# Autodesk Inventor assembly: Assembly1
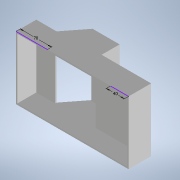
[picture p0: Inventor's stored thumbnail of the model, 180x180]
Saved by Autodesk Inventor 2022 (Build 260153000, 153)
## iProperties
Created: 2021-12-16
Part Number: Assembly1
Document SubType Name: Assembly
Designer: keemi
Author: keemi
## Documents named in this file (9)
- C:\Users\keemi\OneDrive\Bureaublad\repo's\projecten\Auto\modellen\inventor\auto moddel\Assembly1.iam
- C:\Users\keemi\OneDrive\Bureaublad\repo's\projecten\Auto\modellen\inventor\auto moddel\zijkant.ipt
- C:\Users\keemi\OneDrive\Bureaublad\repo's\projecten\Auto\modellen\inventor\auto moddel\onderkant.ipt
- C:\Users\keemi\OneDrive\Bureaublad\repo's\projecten\Auto\modellen\inventor\auto moddel\voorkant.ipt
- C:\Users\keemi\OneDrive\Bureaublad\repo's\projecten\Auto\modellen\inventor\auto moddel\achterkant.ipt
- C:\Users\keemi\OneDrive\Bureaublad\repo's\projecten\Auto\modellen\inventor\auto moddel\motorkap.ipt
- C:\Users\keemi\OneDrive\Bureaublad\repo's\projecten\Auto\modellen\inventor\auto moddel\achterruit.ipt
- C:\Users\keemi\OneDrive\Bureaublad\repo's\projecten\Auto\modellen\inventor\auto moddel\bak.ipt
- C:\Users\keemi\OneDrive\Bureaublad\repo's\projecten\Auto\modellen\inventor\auto moddel\DAK.ipt
## Components (9 placed, 8 different names)
1. zijkant:1 — Flush:11, Flush:12, Flush:13, Flush:14, Flush:15, Flush:16, Flush:18, Flush:20, Flush:24
2. onderkant:1 — Flush:3, Flush:4, Flush:5, Flush:8, Flush:11, Flush:12
3. zijkant:2 — Flush:3, Flush:4, Flush:5, Flush:9, Flush:10, Mate:1, Flush:23, Flush:25
4. voorkant:1 — Flush:8, Flush:9, Flush:10, Flush:13, Flush:17, Flush:19
5. achterkant:1 — Flush:14, Flush:15, Flush:16
6. motorkap:1 — Flush:17, Flush:18, Flush:19
7. achterruit:1 — Flush:20, Flush:21, Flush:22, Flush:23, Flush:26
8. bak:1 — Flush:21, Flush:22, Mate:1
9. DAK:1 — Flush:24, Flush:25, Flush:26
## Relationships (23: Flush 22, Mate 1)
- Flush:3: onderkant:1 ↔ zijkant:2
- Flush:4: onderkant:1 ↔ zijkant:2
- Flush:5: onderkant:1 ↔ zijkant:2
- Flush:8: onderkant:1 ↔ voorkant:1
- Flush:9: zijkant:2 ↔ voorkant:1
- Flush:10: zijkant:2 ↔ voorkant:1
- Flush:11: zijkant:1 ↔ onderkant:1
- Flush:12: zijkant:1 ↔ onderkant:1
- Flush:13: zijkant:1 ↔ voorkant:1
- Flush:14: zijkant:1 ↔ achterkant:1
- Flush:15: zijkant:1 ↔ achterkant:1
- Flush:16: zijkant:1 ↔ achterkant:1
- Flush:17: voorkant:1 ↔ motorkap:1
- Flush:18: zijkant:1 ↔ motorkap:1
- Flush:19: voorkant:1 ↔ motorkap:1
- Flush:20: zijkant:1 ↔ achterruit:1
- Flush:21: achterruit:1 ↔ bak:1
- Flush:22: achterruit:1 ↔ bak:1
- Mate:1: zijkant:2 ↔ bak:1
- Flush:23: zijkant:2 ↔ achterruit:1
- Flush:24: zijkant:1 ↔ DAK:1
- Flush:25: zijkant:2 ↔ DAK:1
- Flush:26: achterruit:1 ↔ DAK:1
